# Autodesk Inventor assembly: adapter
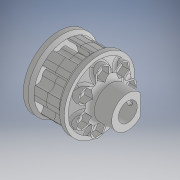
[picture p0: Inventor's stored thumbnail of the model, 180x180]
Saved by Autodesk Inventor 2022 (Build 260153000, 153)
## iProperties
Created: 2023-01-08
Part Number: adapter
Document SubType Name: Assembly
Designer: Иван Петров
Author: Иван Петров
## Documents named in this file (3)
- C:\Users\Ivan Petrov\Documents\GitHub\OmniBot\design\standart_components\VEX Meccanum wheel\adapter.iam
- C:\Users\Ivan Petrov\Documents\GitHub\OmniBot\design\standart_components\vex_mechanum_adapter.ipt
- C:\Users\Ivan Petrov\Documents\GitHub\OmniBot\design\standart_components\vex_mechanum_adapter (1) зеркальный.ipt
## Components (2 placed, 2 different names)
1. vex_mechanum_adapter:1 — Совмещение:1, Совмещение:2, Совмещение:3, Совмещение:4, Заподлицо:1, Угол:1
2. vex_mechanum_adapter (1) зеркальный:1 — Совмещение:2, Совмещение:3, Совмещение:4
## Relationships (6: Mate 4, Flush 1, Angle 1)
- Совмещение:1 [Mate]: vex_mechanum_adapter:1
- Совмещение:2 [Mate]: vex_mechanum_adapter:1 ↔ vex_mechanum_adapter (1) зеркальный:1
- Совмещение:3 [Mate]: vex_mechanum_adapter:1 ↔ vex_mechanum_adapter (1) зеркальный:1
- Совмещение:4 [Mate]: vex_mechanum_adapter:1 ↔ vex_mechanum_adapter (1) зеркальный:1
- Заподлицо:1 [Flush]: vex_mechanum_adapter:1
- Угол:1 [Angle] (0 deg): vex_mechanum_adapter:1
